# Autodesk Inventor assembly: DOMS ASSEMBLY
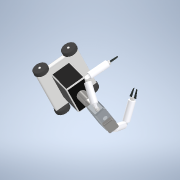
[picture p0: Inventor's stored thumbnail of the model, 180x180]
Saved by Autodesk Inventor 2022 (Build 260153000, 153)
## iProperties
Created: 2021-10-29
Part Number: DOMS ASSEMBLY
Document SubType Name: Assembly
Designer: Mark Maara
Mass: 430070 g
Surface Area: 62993.1 cm^2
Volume: 168993 cm^3
Density: 2.5449 g/cm^3
Author: Mark Maara
## Documents named in this file (17)
- C:\Users\Mark Maara\Documents\Doms2\DOMS ASSEMBLY.iam
- C:\Users\Mark Maara\Documents\Doms2\Shoulder1.ipt
- C:\Users\Mark Maara\Documents\Doms2\Arm1.ipt
- C:\Users\Mark Maara\Documents\Doms2\Chest.ipt
- C:\Users\Mark Maara\Documents\Doms2\Shoulder1_MIR.ipt
- C:\Users\Mark Maara\Documents\Doms2\Arm1_MIR.ipt
- C:\Users\Mark Maara\Documents\Doms2\Camera2.ipt
- C:\Users\Mark Maara\Documents\Doms2\Grip.ipt
- C:\Users\Mark Maara\Documents\Doms2\Stand1.ipt
- C:\Users\Mark Maara\Documents\Doms2\Base Prime.ipt
- C:\Users\Mark Maara\Documents\Doms2\Wheels.ipt
- C:\Users\Mark Maara\Documents\Doms2\DOMS ASSEMBLY\AIP\FEA\ds2rbudr4.fins
- C:\Users\Mark Maara\Documents\Doms2\DOMS ASSEMBLY\AIP\FEA\ds2rbudr4.fsat
- C:\Users\Mark Maara\Documents\Doms2\DOMS ASSEMBLY\AIP\FEA\ds2rbudr4.ftes
- C:\Users\Mark Maara\Documents\Doms2\DOMS ASSEMBLY\AIP\FEA\ds2rbudr4.fwiz
- C:\Users\Mark Maara\Documents\Doms2\DOMS ASSEMBLY\AIP\FEA\ds2shyf9c.fmsh
- C:\Users\Mark Maara\Documents\Doms2\DOMS ASSEMBLY\AIP\FEA\ds2shyf9d.fres
## Components (18 placed, 10 different names)
1. Shoulder1:1 — Rotational:2, Rotational:9
2. Shoulder1:2 — Rotational:1, Rotational:3
3. Arm1:1 — Rotational:1, Rotational:11
4. Arm1:2 — Rotational:2, Rotational:3
5. Chest:1 — Rotational:8, Rotational:9, Rotational:10, Rotational:14
6. Shoulder1_MIR:1 — Rotational:7, Rotational:8
7. Shoulder1_MIR:2 — Rotational:5, Rotational:6
8. Arm1_MIR:1 — Rotational:5, Rotational:12
9. Arm1_MIR:2 — Rotational:6, Rotational:7
10. Camera2:1 — Rotational:10
11. Grip:1 — Rotational:11
12. Grip:2 — Rotational:12
13. Stand1:1 — Rotational:13, Rotational:14
14. Base Prime:1 — Rotational:13, Cylindrical:1, Cylindrical:2, Cylindrical:3, Cylindrical:4
15. Wheels:1 — Cylindrical:2
16. Wheels:2 — Cylindrical:3
17. Wheels:3 — Cylindrical:1
18. Wheels:4 — Cylindrical:4
## Relationships (17: RevoluteJoint 13, CylindricalJoint 4)
- Rotational:1 [RevoluteJoint]: Shoulder1:2 ↔ Arm1:1
- Rotational:2 [RevoluteJoint]: Shoulder1:1 ↔ Arm1:2
- Rotational:3 [RevoluteJoint]: Shoulder1:2 ↔ Arm1:2
- Rotational:5 [RevoluteJoint]: Shoulder1_MIR:2 ↔ Arm1_MIR:1
- Rotational:6 [RevoluteJoint]: Shoulder1_MIR:2 ↔ Arm1_MIR:2
- Rotational:7 [RevoluteJoint]: Shoulder1_MIR:1 ↔ Arm1_MIR:2
- Rotational:8 [RevoluteJoint]: Chest:1 ↔ Shoulder1_MIR:1
- Rotational:9 [RevoluteJoint]: Shoulder1:1 ↔ Chest:1
- Rotational:10 [RevoluteJoint]: Chest:1 ↔ Camera2:1
- Rotational:11 [RevoluteJoint]: Arm1:1 ↔ Grip:1
- Rotational:12 [RevoluteJoint]: Arm1_MIR:1 ↔ Grip:2
- Rotational:13 [RevoluteJoint]: Stand1:1 ↔ Base Prime:1
- Rotational:14 [RevoluteJoint]: Chest:1 ↔ Stand1:1
- Cylindrical:1: Base Prime:1 ↔ Wheels:3
- Cylindrical:2: Base Prime:1 ↔ Wheels:1
- Cylindrical:3: Base Prime:1 ↔ Wheels:2
- Cylindrical:4: Base Prime:1 ↔ Wheels:4
## Named parameters: sa_0 = 1500, sa_1 = 4000
note: some values were not read from the file. Shown as the stored number, unit unknown: "sa_0", "sa_1".
